# Autodesk Inventor assembly: Z_PLATE
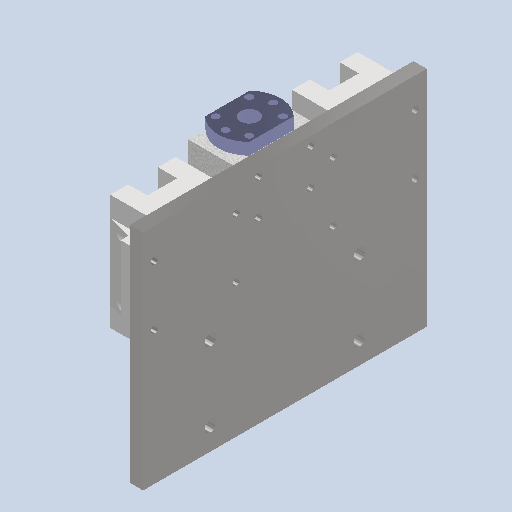
[picture p0: Inventor's stored thumbnail of the model, 512x512]
Saved by Autodesk Inventor 2023 (Build 270158000, 158)
## iProperties
Created: 2022-05-07
Part Number: Z_PLATE
Document SubType Name: Assembly
Designer: plebbb
Author: plebbb
## Documents named in this file (5)
- C:\Users\think\OneDrive\Desktop\CNC_Project\Z_PLATE.iam
- C:\Users\think\OneDrive\Desktop\CNC_Project\HGW20CC_Slider.ipt
- C:\Users\think\OneDrive\Desktop\CNC_Project\Spindle_Mounting_Plate.ipt
- C:\Users\think\OneDrive\Desktop\CNC_Project\DSG12H.ipt
- C:\Users\think\OneDrive\Desktop\CNC_Project\SFU1204_Nut.ipt
## Components (5 placed, 4 different names)
1. HGW20CC_Slider:1
2. HGW20CC_Slider:2
3. Spindle_Mounting_Plate:1
4. DSG12H:1
5. SFU1204_Nut:1
## Relationships (9: Mate 9)
- [Mate]: HGW20CC_Slider:2 ↔ Spindle_Mounting_Plate:1
- [Mate]: HGW20CC_Slider:1 ↔ Spindle_Mounting_Plate:1
- [Mate]: HGW20CC_Slider:1 ↔ Spindle_Mounting_Plate:1
- [Mate]: Spindle_Mounting_Plate:1 ↔ DSG12H:1
- [Mate]: Spindle_Mounting_Plate:1 ↔ DSG12H:1
- [Mate]: Spindle_Mounting_Plate:1 ↔ DSG12H:1
- [Mate]: DSG12H:1 ↔ SFU1204_Nut:1
- [Mate]: DSG12H:1 ↔ SFU1204_Nut:1
- [Mate]: DSG12H:1 ↔ SFU1204_Nut:1
